# Autodesk Inventor assembly: pre_assembly
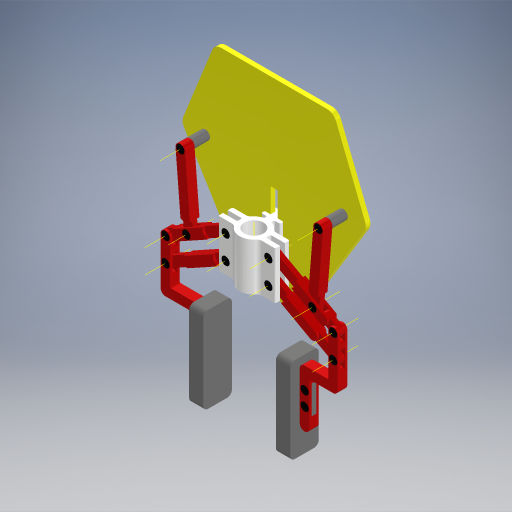
[picture p0: Inventor's stored thumbnail of the model, 512x512]
Saved by Autodesk Inventor 2024.1 (Build 281209000, 209)
## iProperties
Created: 2023-11-07
Part Number: pre_assembly
Document SubType Name: Assembly
Designer: Camilo
Author: Camilo
## Documents named in this file (12)
- D:\Documentos\MEGA\Universidad\2023-2\DinamicaComputacionalDeSistemasMulticuerpo\DinamicaComputacionalSistemasMulticuerpo\Proyecto\CAD\3D\FullAssembly.iam
- D:\Documentos\MEGA\Universidad\2023-2\DinamicaComputacionalDeSistemasMulticuerpo\DinamicaComputacionalSistemasMulticuerpo\Proyecto\CAD\3D\link1_SubAssembly.iam
- D:\Documentos\MEGA\Universidad\2023-2\DinamicaComputacionalDeSistemasMulticuerpo\DinamicaComputacionalSistemasMulticuerpo\Proyecto\CAD\3D\link5_SubAssembly.iam
- D:\Documentos\MEGA\Universidad\2023-2\DinamicaComputacionalDeSistemasMulticuerpo\DinamicaComputacionalSistemasMulticuerpo\Proyecto\CAD\3D\link2.ipt
- D:\Documentos\MEGA\Universidad\2023-2\DinamicaComputacionalDeSistemasMulticuerpo\DinamicaComputacionalSistemasMulticuerpo\Proyecto\CAD\3D\link3.ipt
- D:\Documentos\MEGA\Universidad\2023-2\DinamicaComputacionalDeSistemasMulticuerpo\DinamicaComputacionalSistemasMulticuerpo\Proyecto\CAD\3D\link6_SubAssembly.iam
- D:\Documentos\MEGA\Universidad\2023-2\DinamicaComputacionalDeSistemasMulticuerpo\DinamicaComputacionalSistemasMulticuerpo\Proyecto\CAD\3D\link7_SubAssembly.iam
- D:\Documentos\MEGA\Universidad\2023-2\DinamicaComputacionalDeSistemasMulticuerpo\DinamicaComputacionalSistemasMulticuerpo\Proyecto\CAD\3D\link8.ipt
- D:\Documentos\MEGA\Universidad\2023-2\DinamicaComputacionalDeSistemasMulticuerpo\DinamicaComputacionalSistemasMulticuerpo\Proyecto\CAD\3D\link9.ipt
- D:\Documentos\MEGA\Universidad\2023-2\DinamicaComputacionalDeSistemasMulticuerpo\DinamicaComputacionalSistemasMulticuerpo\Proyecto\CAD\3D\link10_SubAssembly.iam
- D:\Documentos\MEGA\Universidad\2023-2\DinamicaComputacionalDeSistemasMulticuerpo\DinamicaComputacionalSistemasMulticuerpo\Proyecto\CAD\3D\link11_SubAssembly.iam
- link9_SubAssembly.ipt
## Components (10 placed, 10 different names)
1. link1_SubAssembly:1 [sub-assembly] — Mate:1, Mate:2, Insert:1, Insert:2
2. link5_SubAssembly:1 [sub-assembly] — Mate:1, Mate:2, Insert:5, Insert:6, Insert:7, Insert:8
3. link2:1 — Insert:1, Insert:3
4. link3:1 — Insert:2, Insert:4
5. link6_SubAssembly:1 [sub-assembly] — Insert:3, Insert:5, Insert:9
6. link7_SubAssembly:1 [sub-assembly] — Insert:4, Insert:6, Insert:10
7. link8:1 — Insert:7, Insert:11
8. link9:1 — Insert:8, Insert:12
9. link10_SubAssembly:1 [sub-assembly] — Insert:9, Insert:11
10. link11_SubAssembly:1 [sub-assembly] — Insert:10, Insert:12
## Relationships (14: Insert 12, Mate 2)
- Mate:1: link1_SubAssembly:1 ↔ link5_SubAssembly:1
- Mate:2: link1_SubAssembly:1 ↔ link5_SubAssembly:1
- Insert:1: link1_SubAssembly:1 ↔ link2:1
- Insert:2: link1_SubAssembly:1 ↔ link3:1
- Insert:3: link2:1 ↔ link6_SubAssembly:1
- Insert:4: link3:1 ↔ link7_SubAssembly:1
- Insert:5: link5_SubAssembly:1 ↔ link6_SubAssembly:1
- Insert:6: link5_SubAssembly:1 ↔ link7_SubAssembly:1
- Insert:7: link5_SubAssembly:1 ↔ link8:1
- Insert:8: link5_SubAssembly:1 ↔ link9:1
- Insert:9: link6_SubAssembly:1 ↔ link10_SubAssembly:1
- Insert:10: link7_SubAssembly:1 ↔ link11_SubAssembly:1
- Insert:11: link8:1 ↔ link10_SubAssembly:1
- Insert:12: link9:1 ↔ link11_SubAssembly:1
